# Autodesk Inventor assembly: coil
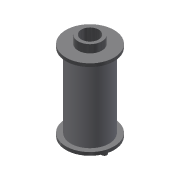
[picture p0: Inventor's stored thumbnail of the model, 180x180]
Saved by Autodesk Inventor 2022 (Build 260148000, 148)
## iProperties
Shininess: 64.0
Length Units: 11272
Angle Units: 11279
Time Units: 11290
Mass Units: 11286
Length Display Precision: 3
Angle Display Precision: 2
Created: 2002-05-01
Part Number: coil
Document SubType Name: Assembly
Designer: Administrator
Density: 0.0
Volumn: 0.0
Area: 0.0
PropertySet Name: Model Information
Control State: 0
Master: False
Checked Out: False
Author: Administrator
## Documents named in this file (3)
- C:\Autodesk Inventor 2022 Advanced Assembly Modeling Practice Files\coil.iam
- C:\Autodesk Inventor 2022 Advanced Assembly Modeling Practice Files\bobbin.ipt
- C:\Autodesk Inventor 2022 Advanced Assembly Modeling Practice Files\coilwire.ipt
## Components (2 placed, 2 different names)
1. bobbin:1 — Insert:1, Mate:1
2. coilwire:1 — Insert:1, Mate:1
## Relationships (2: Insert 1, Mate 1)
- Insert:1: bobbin:1 ↔ coilwire:1
- Mate:1: bobbin:1 ↔ coilwire:1
